# Autodesk Inventor assembly: 51
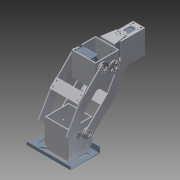
[picture p0: Inventor's stored thumbnail of the model, 180x180]
Saved by Autodesk Inventor 2013 (Build 170138000, 138)
## iProperties
Created: 2014-03-10
Part Number: 51
Document SubType Name: Assembly
Designer: andou
Author: andou
Title: Leg(right)
## Documents named in this file (14)
- C:\Users\andou\Documents\GitHub\Robotics-Project\design\RoboticsProject\project_4\Left_Leg.iam
- C:\Users\andou\Documents\GitHub\Robotics-Project\design\RoboticsProject\project_4\Serial_Case.ipt
- C:\Users\andou\Documents\GitHub\Robotics-Project\design\RoboticsProject\project_4\Generic Parts\KRS-2542HV.ipt
- C:\Users\andou\Documents\GitHub\Robotics-Project\design\RoboticsProject\project_4\Dual_Link_Flame(left).ipt
- C:\Users\andou\Documents\GitHub\Robotics-Project\design\RoboticsProject\project_4\Bracket.ipt
- C:\Users\andou\Documents\GitHub\Robotics-Project\design\RoboticsProject\project_4\Generic Parts\Low_Height_Horn.ipt
- C:\Users\andou\Documents\GitHub\Robotics-Project\design\RoboticsProject\project_4\Free-Horn.iam
- C:\Users\andou\Documents\GitHub\Robotics-Project\design\RoboticsProject\project_4\Parallel_Link_Supporter.ipt
- C:\Users\andou\Documents\GitHub\Robotics-Project\design\RoboticsProject\project_4\Horn-Spacer.ipt
- C:\Users\andou\Documents\GitHub\Robotics-Project\design\RoboticsProject\project_4\Dual_Link_Flame(right).ipt
- C:\Users\andou\Documents\GitHub\Robotics-Project\design\RoboticsProject\project_4\Parallel_Case.ipt
- C:\Users\andou\Documents\GitHub\Robotics-Project\design\RoboticsProject\project_4\Left_Parallel_Case.ipt
- C:\Users\andou\Documents\GitHub\Robotics-Project\design\RoboticsProject\project_4\Left_Sole.ipt
- C:\Users\andou\Documents\GitHub\Robotics-Project\design\RoboticsProject\project_4\Left_Sole_Spacer.ipt
## Components (25 placed, 13 different names)
1. Serial_Case:1 — 挿入:3, 挿入:4, 挿入:25
2. KRS-2542HV:1 — 挿入:3, 挿入:4, 挿入:9
3. KRS-2542HV:2 — 挿入:17, 挿入:98, 挿入:99
4. Dual_Link_Flame(left):3 — 挿入:55, 挿入:56, 挿入:65, 挿入:93, 挿入:104, 挿入:106
5. Dual_Link_Flame(left):4 — 挿入:41, 挿入:54, 挿入:58, 挿入:66, 挿入:87, 挿入:94, 挿入:95, 挿入:105
6. Bracket:1 — 挿入:60, 挿入:61, 挿入:96, 挿入:97, 挿入:109, 挿入:110
7. Low_Height_Horn:1 — 挿入:9, 挿入:60, 挿入:97
8. Low_Height_Horn:2 — 挿入:17, 挿入:68, 挿入:88, 挿入:104
9. Free-Horn:1 [sub-assembly] — 挿入:25, 挿入:61, 挿入:96
10. Free-Horn:2 [sub-assembly] — 挿入:102, 挿入:103, 挿入:108
11. Free-Horn:4 [sub-assembly] — 挿入:41, 挿入:95, 挿入:100, 挿入:105
12. Free-Horn:5 [sub-assembly] — 挿入:54, 挿入:87, 挿入:94
13. Free-Horn:7 [sub-assembly] — 挿入:55, 挿入:83, 挿入:93
14. Parallel_Link_Supporter:1 — 挿入:56, 挿入:65, 挿入:75, 挿入:76
15. Parallel_Link_Supporter:2 — 挿入:58, 挿入:66, 挿入:77, 挿入:78
16. Horn-Spacer:2 — 挿入:68, 挿入:88, 挿入:106
17. Dual_Link_Flame(right):1 — 挿入:75, 挿入:76, 挿入:81, 挿入:92, 挿入:103, 挿入:108
18. Dual_Link_Flame(right):2 — 挿入:77, 挿入:78, 挿入:82, 挿入:86, 挿入:90, 挿入:91, 挿入:107
19. Free-Horn:8 [sub-assembly] — 挿入:81, 挿入:84, 挿入:92
20. Free-Horn:9 [sub-assembly] — 挿入:82, 挿入:90, 挿入:101, 挿入:107
21. Parallel_Case:1 — 挿入:83, 挿入:84, 挿入:85, 挿入:111, 挿入:112
22. Free-Horn:10 [sub-assembly] — 挿入:85, 挿入:86, 挿入:91
23. Left_Parallel_Case:1 — 挿入:98, 挿入:99, 挿入:100, 挿入:101, 挿入:102, 挿入:109, 挿入:110
24. Left_Sole:1 — 挿入:113, 挿入:114
25. Left_Sole_Spacer:1 — 挿入:111, 挿入:112, 挿入:113, 挿入:114
## Relationships (52: Insert 52)
- 挿入:3 [Insert]: Serial_Case:1 ↔ KRS-2542HV:1
- 挿入:4 [Insert]: Serial_Case:1 ↔ KRS-2542HV:1
- 挿入:9 [Insert]: KRS-2542HV:1 ↔ Low_Height_Horn:1
- 挿入:17 [Insert]: KRS-2542HV:2 ↔ Low_Height_Horn:2
- 挿入:25 [Insert]: Serial_Case:1 ↔ Free-Horn:1
- 挿入:41 [Insert]: Dual_Link_Flame(left):4 ↔ Free-Horn:4
- 挿入:54 [Insert]: Dual_Link_Flame(left):4 ↔ Free-Horn:5
- 挿入:55 [Insert]: Dual_Link_Flame(left):3 ↔ Free-Horn:7
- 挿入:56 [Insert]: Dual_Link_Flame(left):3 ↔ Parallel_Link_Supporter:1
- 挿入:58 [Insert]: Dual_Link_Flame(left):4 ↔ Parallel_Link_Supporter:2
- 挿入:60 [Insert]: Bracket:1 ↔ Low_Height_Horn:1
- 挿入:61 [Insert]: Bracket:1 ↔ Free-Horn:1
- 挿入:65 [Insert]: Dual_Link_Flame(left):3 ↔ Parallel_Link_Supporter:1
- 挿入:66 [Insert]: Dual_Link_Flame(left):4 ↔ Parallel_Link_Supporter:2
- 挿入:68 [Insert]: Low_Height_Horn:2 ↔ Horn-Spacer:2
- 挿入:75 [Insert]: Parallel_Link_Supporter:1 ↔ Dual_Link_Flame(right):1
- 挿入:76 [Insert]: Parallel_Link_Supporter:1 ↔ Dual_Link_Flame(right):1
- 挿入:77 [Insert]: Parallel_Link_Supporter:2 ↔ Dual_Link_Flame(right):2
- 挿入:78 [Insert]: Parallel_Link_Supporter:2 ↔ Dual_Link_Flame(right):2
- 挿入:81 [Insert]: Dual_Link_Flame(right):1 ↔ Free-Horn:8
- 挿入:82 [Insert]: Dual_Link_Flame(right):2 ↔ Free-Horn:9
- 挿入:83 [Insert]: Free-Horn:7 ↔ Parallel_Case:1
- 挿入:84 [Insert]: Free-Horn:8 ↔ Parallel_Case:1
- 挿入:85 [Insert]: Parallel_Case:1 ↔ Free-Horn:10
- 挿入:86 [Insert]: Dual_Link_Flame(right):2 ↔ Free-Horn:10
- 挿入:87 [Insert]: Dual_Link_Flame(left):4 ↔ Free-Horn:5
- 挿入:88 [Insert]: Low_Height_Horn:2 ↔ Horn-Spacer:2
- 挿入:90 [Insert]: Dual_Link_Flame(right):2 ↔ Free-Horn:9
- 挿入:91 [Insert]: Dual_Link_Flame(right):2 ↔ Free-Horn:10
- 挿入:92 [Insert]: Dual_Link_Flame(right):1 ↔ Free-Horn:8
- 挿入:93 [Insert]: Dual_Link_Flame(left):3 ↔ Free-Horn:7
- 挿入:94 [Insert]: Dual_Link_Flame(left):4 ↔ Free-Horn:5
- 挿入:95 [Insert]: Dual_Link_Flame(left):4 ↔ Free-Horn:4
- 挿入:96 [Insert]: Bracket:1 ↔ Free-Horn:1
- 挿入:97 [Insert]: Bracket:1 ↔ Low_Height_Horn:1
- 挿入:98 [Insert]: KRS-2542HV:2 ↔ Left_Parallel_Case:1
- 挿入:99 [Insert]: KRS-2542HV:2 ↔ Left_Parallel_Case:1
- 挿入:100 [Insert]: Free-Horn:4 ↔ Left_Parallel_Case:1
- 挿入:101 [Insert]: Free-Horn:9 ↔ Left_Parallel_Case:1
- 挿入:102 [Insert]: Free-Horn:2 ↔ Left_Parallel_Case:1
- 挿入:103 [Insert]: Free-Horn:2 ↔ Dual_Link_Flame(right):1
- 挿入:104 [Insert]: Dual_Link_Flame(left):3 ↔ Low_Height_Horn:2
- 挿入:105 [Insert]: Dual_Link_Flame(left):4 ↔ Free-Horn:4
- 挿入:106 [Insert]: Dual_Link_Flame(left):3 ↔ Horn-Spacer:2
- 挿入:107 [Insert]: Dual_Link_Flame(right):2 ↔ Free-Horn:9
- 挿入:108 [Insert]: Free-Horn:2 ↔ Dual_Link_Flame(right):1
- 挿入:109 [Insert]: Bracket:1 ↔ Left_Parallel_Case:1
- 挿入:110 [Insert]: Bracket:1 ↔ Left_Parallel_Case:1
- 挿入:111 [Insert]: Parallel_Case:1 ↔ Left_Sole_Spacer:1
- 挿入:112 [Insert]: Parallel_Case:1 ↔ Left_Sole_Spacer:1
- 挿入:113 [Insert]: Left_Sole:1 ↔ Left_Sole_Spacer:1
- 挿入:114 [Insert]: Left_Sole:1 ↔ Left_Sole_Spacer:1
